# Autodesk Inventor assembly: quadcopter
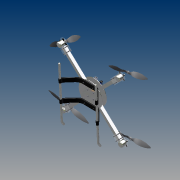
[picture p0: Inventor's stored thumbnail of the model, 180x180]
Saved by Autodesk Inventor 2011 SP1 (Build 150282100, 282)
## iProperties
Created: 2011-07-18
Part Number: quadcopter
Document SubType Name: Assembly
Designer: Nathan
Author: Nathan
## Documents named in this file (19)
- C:\Users\Nathan\Documents\Inventor\Quadcopter\quadcopter - box.iam
- C:\Users\Nathan\Documents\Inventor\Quadcopter\Arm.ipt
- C:\Users\Nathan\Documents\Inventor\Quadcopter\BaseTop.ipt
- C:\Users\Nathan\Documents\Inventor\Quadcopter\BaseBottom.ipt
- C:\Users\Nathan\Documents\Inventor\Quadcopter\MotorMount.iam
- C:\Users\Nathan\Documents\Inventor\Quadcopter\standoffiPart.ipt
- C:\Users\Nathan\Documents\Inventor\Quadcopter\standoffiPart-01.ipt
- C:\Users\Nathan\Documents\Inventor\Quadcopter\standoffiPart-011.ipt
- C:\Users\Nathan\Documents\Inventor\Content Center Files\R2011\en-US\ANSI B18.6.3(26)\ANSI B18.6.3 - 8-32 UNC - 1.25(7).ipt
- C:\Users\Nathan\Documents\Inventor\Content Center Files\R2011\en-US\ANSI B18.6.3(26)\ANSI B18.6.3 - 8-32 UNC - 1.125(7).ipt
- C:\Users\Nathan\Documents\Inventor\Quadcopter\Imported Components\User Library-Arduino Mega\Assembly2.iam
- C:\Users\Nathan\Documents\Inventor\Quadcopter\LandingGear.iam
- C:\Users\Nathan\Documents\Inventor\Quadcopter\Motor.iam
- C:\Users\Nathan\Documents\Inventor\Quadcopter\propeller.iam
- C:\Users\Nathan\Documents\Inventor\Content Center Files\R2011\en-US\ANSI B18.6.3(26)\ANSI B18.6.3 - 6-32 UNC - 0.5625(7).ipt
- C:\Users\Nathan\Documents\Inventor\Quadcopter\PropProtector.ipt
- C:\Users\Nathan\Documents\Inventor\Content Center Files\R2011\en-US\ANSI B18.6.3(26)\ANSI B18.6.3 - 8-32 UNC - 1.375(7).ipt
- C:\Users\Nathan\Documents\Inventor\Content Center Files\R2011\en-US\ANSI B18.6.3(26)\ANSI B18.6.3 - 6-32 UNC - 0.5(7).ipt
- C:\Users\Nathan\Documents\Inventor\Quadcopter\standoffiPart-014.ipt
## Components (41 placed, 17 different names)
1. Arm:1 — Mate:1, Mate:2, Mate:15, Flush:20, Mate:20, Flush:27, Mate:66, Mate:68
2. Arm:2 — Mate:5, Mate:6, Flush:21, Mate:21, Mate:38, Flush:25, Mate:74, Mate:76
3. Arm:3 — Mate:3, Mate:4, Flush:22, Mate:22, Flush:24, Mate:63, Mate:70, Mate:72
4. Arm:4 — Mate:7, Mate:8, Flush:23, Mate:23, Flush:26, Mate:78, Mate:79, Mate:97
5. BaseTop:1 — Mate:1, Mate:2, Mate:3, Mate:4, Mate:5, Mate:6, Mate:7, Mate:8, Mate:13, Mate:14, Mate:16, Mate:18, Mate:24, Mate:25, Mate:46, Mate:47, Mate:48, Mate:49, Mate:98, Angle:1, Flush:28, Flush:29
6. BaseBottom:1 — Mate:13, Mate:14, Mate:15, Mate:17, Mate:19, Mate:26, Mate:27, Mate:38, Mate:50, Mate:51, Mate:52, Mate:53, Mate:63, Mate:97, Mate:113, Mate:114, Mate:115, Mate:148, Mate:149, Mate:150, Mate:151, Mate:152, Mate:153, Mate:154, Mate:155
7. Cross Recessed Pan Head Machine Screw - Type II - Inch No. 8 - 32 - 1 1/4:1 — Mate:16, Mate:17, Mate:65
8. Cross Recessed Pan Head Machine Screw - Type II - Inch No. 8 - 32 - 1 1/8:2 — Mate:18, Mate:19, Mate:67
9. Cross Recessed Pan Head Machine Screw - Type II - Inch No. 8 - 32 - 1 1/4:7 — Mate:24, Mate:26, Mate:69
10. Cross Recessed Pan Head Machine Screw - Type II - Inch No. 8 - 32 - 1 1/8:3 — Mate:25, Mate:27, Mate:71
11. MotorMount:1 [sub-assembly] — Flush:20, Mate:20, Flush:27, Mate:136, Mate:137
12. MotorMount:2 [sub-assembly] — Flush:21, Mate:21, Flush:25, Mate:140, Mate:141
13. MotorMount:3 [sub-assembly] — Flush:22, Mate:22, Flush:24, Mate:142, Mate:143
14. MotorMount:4 [sub-assembly] — Flush:23, Mate:23, Flush:26, Mate:138, Mate:139
15. Cross Recessed Pan Head Machine Screw - Type II - Inch No. 8 - 32 - 1 3/8:1 — Mate:46, Mate:51, Mate:75
16. Cross Recessed Pan Head Machine Screw - Type II - Inch No. 8 - 32 - 1 1/8:4 — Mate:48, Mate:52, Mate:77
17. Cross Recessed Pan Head Machine Screw - Type II - Inch No. 8 - 32 - 1 1/4:2 — Mate:49, Mate:53, Mate:80
18. Cross Recessed Pan Head Machine Screw - Type II - Inch No. 8 - 32 - 1 1/8:1 — Mate:47, Mate:50, Mate:73
19. standoffiPart-01:9 — Mate:65, Mate:66
20. standoffiPart-01:10 — Mate:69, Mate:70
21. standoffiPart-01:11 — Mate:71, Mate:72
22. standoffiPart-01:12 — Mate:67, Mate:68
23. standoffiPart-011:13 — Mate:73, Mate:74
24. standoffiPart-014:14 — Mate:75, Mate:76
25. standoffiPart-011:15 — Mate:79, Mate:80
26. standoffiPart-011:16 — Mate:77, Mate:78, Mate:98
27. Assembly2:1 [sub-assembly] — Angle:1
28. LandingGear:1 [sub-assembly] — Mate:113, Mate:114, Mate:115
29. Motor:1 [sub-assembly] — Mate:136, Mate:137, Mate:146
30. Motor:2 [sub-assembly] — Mate:140, Mate:141, Mate:145
31. Motor:3 [sub-assembly] — Mate:142, Mate:143, Mate:144, Mate:156
32. Motor:4 [sub-assembly] — Mate:138, Mate:139, Mate:147
33. propeller:1 [sub-assembly] — Mate:144
34. propeller:2 [sub-assembly] — Mate:145
35. propeller:3 [sub-assembly] — Mate:146
36. propeller:4 [sub-assembly] — Mate:147
37. Cross Recessed Pan Head Machine Screw - Type II - Inch No. 6 - 32 - 1/2:1 — Mate:148, Mate:149
38. Cross Recessed Pan Head Machine Screw - Type II - Inch No. 6 - 32 - 9/16:4 — Mate:154, Mate:155
39. Cross Recessed Pan Head Machine Screw - Type II - Inch No. 6 - 32 - 9/16:3 — Mate:152, Mate:153
40. Cross Recessed Pan Head Machine Screw - Type II - Inch No. 6 - 32 - 9/16:1 — Mate:150, Mate:151
41. PropProtector:1 — Flush:28, Flush:29, Mate:156
## Relationships (86: Mate 75, Flush 10, Angle 1)
- Mate:1: Arm:1 ↔ BaseTop:1
- Mate:2: Arm:1 ↔ BaseTop:1
- Mate:3: Arm:3 ↔ BaseTop:1
- Mate:4: Arm:3 ↔ BaseTop:1
- Mate:5: Arm:2 ↔ BaseTop:1
- Mate:6: Arm:2 ↔ BaseTop:1
- Mate:7: Arm:4 ↔ BaseTop:1
- Mate:8: Arm:4 ↔ BaseTop:1
- Mate:13: BaseTop:1 ↔ BaseBottom:1
- Mate:14: BaseTop:1 ↔ BaseBottom:1
- Mate:15: Arm:1 ↔ BaseBottom:1
- Mate:16: BaseTop:1 ↔ Cross Recessed Pan Head Machine Screw - Type II - Inch No. 8 - 32 - 1 1/4:1
- Mate:17: BaseBottom:1 ↔ Cross Recessed Pan Head Machine Screw - Type II - Inch No. 8 - 32 - 1 1/4:1
- Mate:18: BaseTop:1 ↔ Cross Recessed Pan Head Machine Screw - Type II - Inch No. 8 - 32 - 1 1/8:2
- Mate:19: BaseBottom:1 ↔ Cross Recessed Pan Head Machine Screw - Type II - Inch No. 8 - 32 - 1 1/8:2
- Flush:20: Arm:1 ↔ MotorMount:1
- Mate:20: Arm:1 ↔ MotorMount:1
- Flush:21: Arm:2 ↔ MotorMount:2
- Mate:21: Arm:2 ↔ MotorMount:2
- Flush:22: Arm:3 ↔ MotorMount:3
- Mate:22: Arm:3 ↔ MotorMount:3
- Flush:23: Arm:4 ↔ MotorMount:4
- Mate:23: Arm:4 ↔ MotorMount:4
- Mate:24: BaseTop:1 ↔ Cross Recessed Pan Head Machine Screw - Type II - Inch No. 8 - 32 - 1 1/4:7
- Mate:25: BaseTop:1 ↔ Cross Recessed Pan Head Machine Screw - Type II - Inch No. 8 - 32 - 1 1/8:3
- Mate:26: BaseBottom:1 ↔ Cross Recessed Pan Head Machine Screw - Type II - Inch No. 8 - 32 - 1 1/4:7
- Mate:27: BaseBottom:1 ↔ Cross Recessed Pan Head Machine Screw - Type II - Inch No. 8 - 32 - 1 1/8:3
- Mate:38: Arm:2 ↔ BaseBottom:1
- Flush:24: Arm:3 ↔ MotorMount:3
- Flush:25: Arm:2 ↔ MotorMount:2
- Flush:26: Arm:4 ↔ MotorMount:4
- Flush:27: Arm:1 ↔ MotorMount:1
- Mate:46: BaseTop:1 ↔ Cross Recessed Pan Head Machine Screw - Type II - Inch No. 8 - 32 - 1 3/8:1
- Mate:47: BaseTop:1 ↔ Cross Recessed Pan Head Machine Screw - Type II - Inch No. 8 - 32 - 1 1/8:1
- Mate:48: BaseTop:1 ↔ Cross Recessed Pan Head Machine Screw - Type II - Inch No. 8 - 32 - 1 1/8:4
- Mate:49: BaseTop:1 ↔ Cross Recessed Pan Head Machine Screw - Type II - Inch No. 8 - 32 - 1 1/4:2
- Mate:50: BaseBottom:1 ↔ Cross Recessed Pan Head Machine Screw - Type II - Inch No. 8 - 32 - 1 1/8:1
- Mate:51: BaseBottom:1 ↔ Cross Recessed Pan Head Machine Screw - Type II - Inch No. 8 - 32 - 1 3/8:1
- Mate:52: BaseBottom:1 ↔ Cross Recessed Pan Head Machine Screw - Type II - Inch No. 8 - 32 - 1 1/8:4
- Mate:53: BaseBottom:1 ↔ Cross Recessed Pan Head Machine Screw - Type II - Inch No. 8 - 32 - 1 1/4:2
- Mate:63: Arm:3 ↔ BaseBottom:1
- Mate:65: Cross Recessed Pan Head Machine Screw - Type II - Inch No. 8 - 32 - 1 1/4:1 ↔ standoffiPart-01:9
- Mate:66: Arm:1 ↔ standoffiPart-01:9
- Mate:67: Cross Recessed Pan Head Machine Screw - Type II - Inch No. 8 - 32 - 1 1/8:2 ↔ standoffiPart-01:12
- Mate:68: Arm:1 ↔ standoffiPart-01:12
- Mate:69: Cross Recessed Pan Head Machine Screw - Type II - Inch No. 8 - 32 - 1 1/4:7 ↔ standoffiPart-01:10
- Mate:70: Arm:3 ↔ standoffiPart-01:10
- Mate:71: Cross Recessed Pan Head Machine Screw - Type II - Inch No. 8 - 32 - 1 1/8:3 ↔ standoffiPart-01:11
- Mate:72: Arm:3 ↔ standoffiPart-01:11
- Mate:73: Cross Recessed Pan Head Machine Screw - Type II - Inch No. 8 - 32 - 1 1/8:1 ↔ standoffiPart-011:13
- Mate:74: Arm:2 ↔ standoffiPart-011:13
- Mate:75: Cross Recessed Pan Head Machine Screw - Type II - Inch No. 8 - 32 - 1 3/8:1 ↔ standoffiPart-014:14
- Mate:76: Arm:2 ↔ standoffiPart-014:14
- Mate:77: Cross Recessed Pan Head Machine Screw - Type II - Inch No. 8 - 32 - 1 1/8:4 ↔ standoffiPart-011:16
- Mate:78: Arm:4 ↔ standoffiPart-011:16
- Mate:79: Arm:4 ↔ standoffiPart-011:15
- Mate:80: Cross Recessed Pan Head Machine Screw - Type II - Inch No. 8 - 32 - 1 1/4:2 ↔ standoffiPart-011:15
- Mate:97: Arm:4 ↔ BaseBottom:1
- Mate:98: BaseTop:1 ↔ standoffiPart-011:16
- Angle:1 (0 deg): BaseTop:1 ↔ Assembly2:1
- Mate:113: BaseBottom:1 ↔ LandingGear:1
- Mate:114: BaseBottom:1 ↔ LandingGear:1
- Mate:115 (3.175 mm): BaseBottom:1 ↔ LandingGear:1
- Mate:136: MotorMount:1 ↔ Motor:1
- Mate:137: MotorMount:1 ↔ Motor:1
- Mate:138: MotorMount:4 ↔ Motor:4
- Mate:139: MotorMount:4 ↔ Motor:4
- Mate:140: MotorMount:2 ↔ Motor:2
- Mate:141: MotorMount:2 ↔ Motor:2
- Mate:142: MotorMount:3 ↔ Motor:3
- Mate:143: MotorMount:3 ↔ Motor:3
- Mate:144: Motor:3 ↔ propeller:1
- Mate:145: Motor:2 ↔ propeller:2
- Mate:146: Motor:1 ↔ propeller:3
- Mate:147: Motor:4 ↔ propeller:4
- Mate:148: BaseBottom:1 ↔ Cross Recessed Pan Head Machine Screw - Type II - Inch No. 6 - 32 - 1/2:1
- Mate:149: BaseBottom:1 ↔ Cross Recessed Pan Head Machine Screw - Type II - Inch No. 6 - 32 - 1/2:1
- Mate:150: BaseBottom:1 ↔ Cross Recessed Pan Head Machine Screw - Type II - Inch No. 6 - 32 - 9/16:1
- Mate:151: BaseBottom:1 ↔ Cross Recessed Pan Head Machine Screw - Type II - Inch No. 6 - 32 - 9/16:1
- Mate:152: BaseBottom:1 ↔ Cross Recessed Pan Head Machine Screw - Type II - Inch No. 6 - 32 - 9/16:3
- Mate:153: BaseBottom:1 ↔ Cross Recessed Pan Head Machine Screw - Type II - Inch No. 6 - 32 - 9/16:3
- Mate:154: BaseBottom:1 ↔ Cross Recessed Pan Head Machine Screw - Type II - Inch No. 6 - 32 - 9/16:4
- Mate:155: BaseBottom:1 ↔ Cross Recessed Pan Head Machine Screw - Type II - Inch No. 6 - 32 - 9/16:4
- Flush:28: BaseTop:1 ↔ PropProtector:1
- Flush:29: BaseTop:1 ↔ PropProtector:1
- Mate:156: Motor:3 ↔ PropProtector:1
